# Autodesk Inventor assembly: KC-362-30
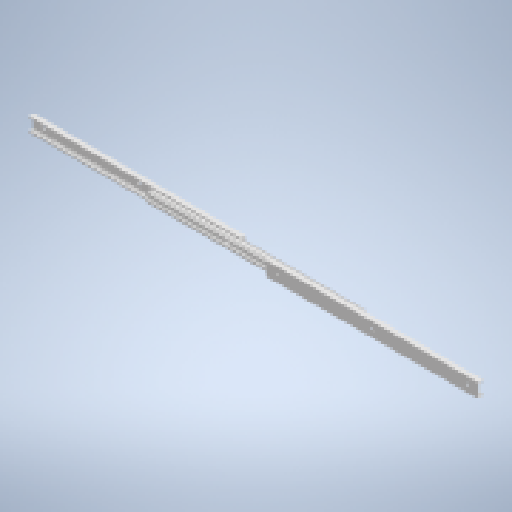
[picture p0: Inventor's stored thumbnail of the model, 512x512]
Saved by Autodesk Inventor 2023 (Build 270158000, 158)
## iProperties
Created: 2022-09-07
Part Number: KC-362-30
Document SubType Name: Assembly
Designer: deli
Author: deli
## Documents named in this file (3)
- C:\Users\deli\OneDrive - Eastside Preparatory School\FTC\8103-power-play\CAD\FTC-parts\KC-362-30.iam
- C:\Users\deli\OneDrive - Eastside Preparatory School\FTC\8103-power-play\CAD\Outside.ipt
- C:\Users\deli\OneDrive - Eastside Preparatory School\FTC\8103-power-play\CAD\FTC-parts\KC-362-30 Middle.ipt
## Components (3 placed, 2 different names)
1. Outside:1
2. KC-362-30 Middle:1
3. Outside:2
## Relationships (5: Mate 4, Flush 1)
- [Mate]: Outside:1 ↔ KC-362-30 Middle:1
- [Mate]: Outside:1 ↔ KC-362-30 Middle:1
- [Mate]: KC-362-30 Middle:1 ↔ Outside:2
- [Mate]: KC-362-30 Middle:1 ↔ Outside:2
- [Flush]: Outside:1 ↔ KC-362-30 Middle:1
## Named parameters: d12_d3 = 0 mm, d13_d4 = 0 mm, d14_d5 = 0 mm, d15_d6 = 0 mm
